# Autodesk Inventor assembly: 360mmPost
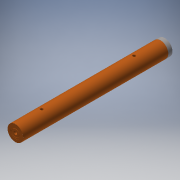
[picture p0: Inventor's stored thumbnail of the model, 180x180]
Saved by Autodesk Inventor 2016 (Build 200138000, 138)
## iProperties
Created: 2016-04-09
Part Number: 360mmPost
Document SubType Name: Assembly
Designer: sims01
Author: sims01
## Documents named in this file (3)
- H:\Documents\LSFM_3\setup\mechanical\design\lsfm3_mechDesignMar16\360mmPost.iam
- H:\Documents\LSFM_3\setup\mechanical\design\lsfm3_mechDesignMar16\350mmMountingPost.ipt
- H:\Documents\LSFM_3\setup\mechanical\design\lsfm3_mechDesignMar16\10mmPostSpacer.ipt
## Components (2 placed, 2 different names)
1. 350mmMountingPost:1 — Rotational:1
2. 10mmPostSpacer:1 — Rotational:1
## Relationships (1: RevoluteJoint 1)
- Rotational:1 [RevoluteJoint]: 350mmMountingPost:1 ↔ 10mmPostSpacer:1
